# Autodesk Inventor assembly: zlozenie_kompetne
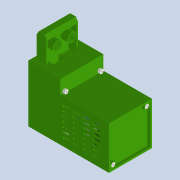
[picture p0: Inventor's stored thumbnail of the model, 180x180]
Saved by Autodesk Inventor 2021 (Build 250183000, 183)
## iProperties
Created: 2025-11-29
Part Number: zlozenie_kompetne
Document SubType Name: Assembly
Designer: huber
Author: huber
## Documents named in this file (13)
- C:\Users\huber\OneDrive\Pulpit\hackaton BHL\BHL 2025\zlozenie_kompetne.iam
- C:\Users\huber\OneDrive\Pulpit\hackaton BHL\BHL 2025\KY-015.ipt
- C:\Users\huber\OneDrive\Pulpit\hackaton BHL\BHL 2025\PCB Prototype( 80X60 ).ipt
- C:\Users\huber\OneDrive\Pulpit\hackaton BHL\BHL 2025\obudowa.ipt
- C:\Users\huber\OneDrive\Pulpit\hackaton BHL\BHL 2025\pokrywa_obudowa.ipt
- C:\Users\huber\OneDrive\Pulpit\hackaton BHL\BHL 2025\Drawer.iam
- C:\Users\huber\Downloads\Solar Panel.ipt
- C:\Users\huber\OneDrive\Pulpit\hackaton BHL\BHL 2025\MQ2 Gas Sensor.ipt
- C:\Users\huber\OneDrive\Pulpit\hackaton BHL\BHL 2025\TP4056_Charging_Module_Type_C.iam
- C:\Users\huber\OneDrive\Pulpit\hackaton BHL\BHL 2025\ESP32-C3 supermini v5.iam
- C:\Users\huber\OneDrive\Pulpit\hackaton BHL\BHL 2025\U1V11F3, Pololu 3.3V Step-Up Voltage Regulator_TOP.iam
- C:\Users\huber\OneDrive\Dokumenty\Inventor\Content Center Files\R2021\en-US\ISO 4762(2)\ISO 4762 - M4 x 16ISO.ipt
- C:\Users\huber\OneDrive\Dokumenty\Inventor\Content Center Files\R2021\en-US\ISO 4762(2)\ISO 4762 - M4 x 12ISO.ipt
## Components (16 placed, 12 different names)
1. KY-015:1 — Angle:1, Mate:3, Mate:17
2. PCB Prototype( 80X60 ):1 — Mate:1, Angle:1, Mate:3, Mate:14, Mate:15, Flush:2, Angle:2, Mate:16, Mate:17, Insert:1, Insert:2, Insert:3
3. obudowa:1 — Mate:1, Mate:4, Mate:5, Mate:6, Mate:8, Mate:9, Mate:13, Flush:2, Angle:3, Angle:4, Angle:5, Insert:4, Insert:5
4. pokrywa_obudowa:1 — Mate:4, Mate:5, Mate:6, Mate:15, Insert:8, Insert:9
5. Drawer:1 [sub-assembly] — Mate:8, Mate:9, Mate:11, Flush:1, Mate:12, Mate:13, Insert:6, Insert:7
6. Solar Panel:1 — Mate:11, Flush:1, Mate:12
7. MQ2 Gas Sensor:1 — Mate:14, Angle:2, Mate:16
8. TP4056_Charging_Module_Type_C:1 [sub-assembly] — Insert:1, Angle:3
9. ESP32-C3 supermini v5:1 [sub-assembly] — Insert:2, Angle:4
10. U1V11F3, Pololu 3.3V Step-Up Voltage Regulator_TOP:1 [sub-assembly] — Insert:3, Angle:5
11. ISO 4762 M4 x 16:1 — Insert:4
12. ISO 4762 M4 x 16:2 — Insert:5
13. ISO 4762 M4 x 16:3 — Insert:6
14. ISO 4762 M4 x 16:4 — Insert:7
15. ISO 4762 M4 x 12:1 — Insert:8
16. ISO 4762 M4 x 12:2 — Insert:9
## Relationships (30: Mate 14, Insert 9, Angle 5, Flush 2)
- Mate:1 (0.25 mm): PCB Prototype( 80X60 ):1 ↔ obudowa:1
- Angle:1 (0 deg): KY-015:1 ↔ PCB Prototype( 80X60 ):1
- Mate:3: KY-015:1 ↔ PCB Prototype( 80X60 ):1
- Mate:4: obudowa:1 ↔ pokrywa_obudowa:1
- Mate:5: obudowa:1 ↔ pokrywa_obudowa:1
- Mate:6: obudowa:1 ↔ pokrywa_obudowa:1
- Mate:8: obudowa:1 ↔ Drawer:1
- Mate:9: obudowa:1 ↔ Drawer:1
- Mate:11: Drawer:1 ↔ Solar Panel:1
- Flush:1 (4.723 mm): Drawer:1 ↔ Solar Panel:1
- Mate:12: Drawer:1 ↔ Solar Panel:1
- Mate:13: obudowa:1 ↔ Drawer:1
- Mate:14: PCB Prototype( 80X60 ):1 ↔ MQ2 Gas Sensor:1
- Mate:15: PCB Prototype( 80X60 ):1 ↔ pokrywa_obudowa:1
- Flush:2 (36.7 mm): PCB Prototype( 80X60 ):1 ↔ obudowa:1
- Angle:2 (0 deg): PCB Prototype( 80X60 ):1 ↔ MQ2 Gas Sensor:1
- Mate:16 (-5 mm): PCB Prototype( 80X60 ):1 ↔ MQ2 Gas Sensor:1
- Mate:17: KY-015:1 ↔ PCB Prototype( 80X60 ):1
- Insert:1: PCB Prototype( 80X60 ):1 ↔ TP4056_Charging_Module_Type_C:1
- Angle:3 (0 deg): obudowa:1 ↔ TP4056_Charging_Module_Type_C:1
- Insert:2: PCB Prototype( 80X60 ):1 ↔ ESP32-C3 supermini v5:1
- Angle:4 (90 deg): obudowa:1 ↔ ESP32-C3 supermini v5:1
- Insert:3: PCB Prototype( 80X60 ):1 ↔ U1V11F3, Pololu 3.3V Step-Up Voltage Regulator_TOP:1
- Angle:5 (180 deg): obudowa:1 ↔ U1V11F3, Pololu 3.3V Step-Up Voltage Regulator_TOP:1
- Insert:4: obudowa:1 ↔ ISO 4762 M4 x 16:1
- Insert:5: obudowa:1 ↔ ISO 4762 M4 x 16:2
- Insert:6: Drawer:1 ↔ ISO 4762 M4 x 16:3
- Insert:7: Drawer:1 ↔ ISO 4762 M4 x 16:4
- Insert:8: pokrywa_obudowa:1 ↔ ISO 4762 M4 x 12:1
- Insert:9: pokrywa_obudowa:1 ↔ ISO 4762 M4 x 12:2
